# Autodesk Inventor assembly: 101
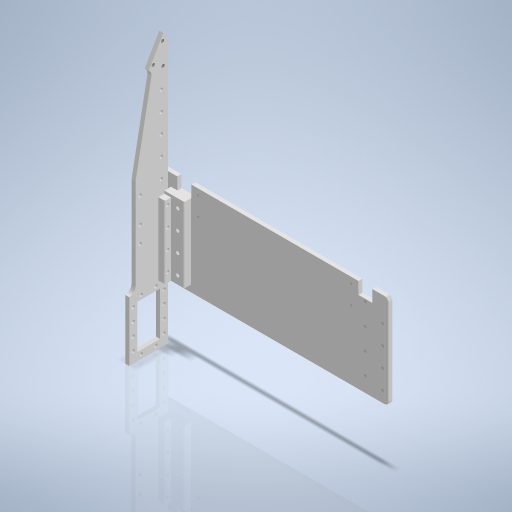
[picture p0: Inventor's stored thumbnail of the model, 512x512]
Saved by Autodesk Inventor 2024 (Build 280153000, 153)
## iProperties
Created: 2024-06-10
Part Number: 101
Document SubType Name: Assembly
Designer: ffogue
Author: ffogue
## Documents named in this file (4)
- C:\Users\ffogue\OneDrive - MuM - OM\Dokumente\Inventor\Paddle\101.iam
- C:\Users\ffogue\OneDrive - MuM - OM\Dokumente\Inventor\Paddle\1011.ipt
- C:\Users\ffogue\OneDrive - MuM - OM\Dokumente\Inventor\Paddle\1014.ipt
- C:\Users\ffogue\OneDrive - MuM - OM\Dokumente\Inventor\Paddle\1012.ipt
## Components (3 placed, 3 different names)
1. 1011:1 — Einfügen:1
2. 1014:1 — Einfügen:1, Einfügen:2
3. 1012:1 — Einfügen:2
## Relationships (2: Insert 2)
- Einfügen:1 [Insert]: 1011:1 ↔ 1014:1
- Einfügen:2 [Insert]: 1014:1 ↔ 1012:1
